# Autodesk Inventor assembly: 射出_骨組み
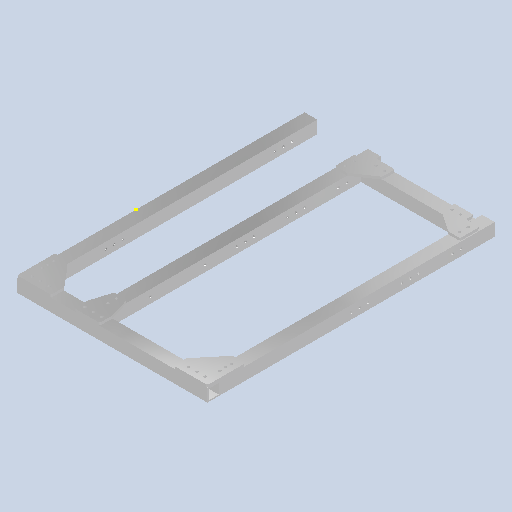
[picture p0: Inventor's stored thumbnail of the model, 512x512]
Saved by Autodesk Inventor 2023 (Build 270158000, 158)
## iProperties
Created: 2022-04-24
Part Number: 射出_骨組み
Document SubType Name: Assembly
Designer: yuta
Author: yuta
## Documents named in this file (9)
- C:\Users\yuta\Documents\NHK\射出_骨組み.iam
- C:\Users\yuta\Documents\NHK\射出_角柱2.ipt
- C:\Users\yuta\Documents\NHK\射出_角柱5.ipt
- C:\Users\yuta\Documents\NHK\射出_角柱4.ipt
- C:\Users\yuta\Documents\NHK\射出_角柱3.ipt
- C:\Users\yuta\Documents\NHK\射出_固定3.ipt
- C:\Users\yuta\Documents\NHK\射出_固定5.ipt
- C:\Users\yuta\Documents\NHK\射出_固定4.ipt
- C:\Users\yuta\Documents\NHK\射出_角柱9.ipt
## Components (10 placed, 8 different names)
1. 射出_角柱2:1 — メイト:18, メイト:19, メイト:20, メイト:21, メイト:25, メイト:26, メイト:27
2. 射出_角柱5:1 — メイト:14, メイト:15, フラッシュ:3, メイト:16, メイト:17, フラッシュ:4
3. 射出_角柱4:1 — メイト:1, フラッシュ:1, フラッシュ:2, メイト:5, メイト:6, メイト:22, メイト:23, メイト:24, メイト:29
4. 射出_角柱3:1 — メイト:1, フラッシュ:1, フラッシュ:2, メイト:2, メイト:3, メイト:4, メイト:7, メイト:8, メイト:9, メイト:10, メイト:11, メイト:12, メイト:13, メイト:15, フラッシュ:4, メイト:19
5. 射出_固定3:1 — メイト:11, メイト:12, メイト:13, メイト:14, フラッシュ:3, メイト:16, メイト:17
6. 射出_固定3:2 — メイト:2, メイト:3, メイト:4, メイト:5, メイト:6
7. 射出_固定5:1 — メイト:7, メイト:8, メイト:9, メイト:10, メイト:18, メイト:20, メイト:21
8. 射出_固定4:1 — メイト:22, メイト:23, メイト:24, メイト:28, メイト:30, メイト:31
9. 射出_固定4:2 — メイト:25, メイト:26, メイト:27, メイト:32, メイト:33
10. 射出_角柱9:1 — メイト:28, メイト:29, メイト:30, メイト:31, メイト:32, メイト:33
## Relationships (37: Mate 33, Flush 4)
- メイト:1 [Mate]: 射出_角柱4:1 ↔ 射出_角柱3:1
- フラッシュ:1 [Flush]: 射出_角柱4:1 ↔ 射出_角柱3:1
- フラッシュ:2 [Flush]: 射出_角柱4:1 ↔ 射出_角柱3:1
- メイト:2 [Mate]: 射出_角柱3:1 ↔ 射出_固定3:2
- メイト:3 [Mate]: 射出_角柱3:1 ↔ 射出_固定3:2
- メイト:4 [Mate]: 射出_角柱3:1 ↔ 射出_固定3:2
- メイト:5 [Mate]: 射出_角柱4:1 ↔ 射出_固定3:2
- メイト:6 [Mate]: 射出_角柱4:1 ↔ 射出_固定3:2
- メイト:7 [Mate]: 射出_角柱3:1 ↔ 射出_固定5:1
- メイト:8 [Mate]: 射出_角柱3:1 ↔ 射出_固定5:1
- メイト:9 [Mate]: 射出_角柱3:1 ↔ 射出_固定5:1
- メイト:10 [Mate]: 射出_角柱3:1 ↔ 射出_固定5:1
- メイト:11 [Mate]: 射出_角柱3:1 ↔ 射出_固定3:1
- メイト:12 [Mate]: 射出_角柱3:1 ↔ 射出_固定3:1
- メイト:13 [Mate]: 射出_角柱3:1 ↔ 射出_固定3:1
- メイト:14 [Mate]: 射出_角柱5:1 ↔ 射出_固定3:1
- メイト:15 [Mate]: 射出_角柱5:1 ↔ 射出_角柱3:1
- フラッシュ:3 [Flush]: 射出_角柱5:1 ↔ 射出_固定3:1
- メイト:16 [Mate]: 射出_角柱5:1 ↔ 射出_固定3:1
- メイト:17 [Mate]: 射出_角柱5:1 ↔ 射出_固定3:1
- フラッシュ:4 [Flush]: 射出_角柱5:1 ↔ 射出_角柱3:1
- メイト:18 [Mate]: 射出_角柱2:1 ↔ 射出_固定5:1
- メイト:19 [Mate]: 射出_角柱2:1 ↔ 射出_角柱3:1
- メイト:20 [Mate]: 射出_角柱2:1 ↔ 射出_固定5:1
- メイト:21 [Mate]: 射出_角柱2:1 ↔ 射出_固定5:1
- メイト:22 [Mate]: 射出_角柱4:1 ↔ 射出_固定4:1
- メイト:23 [Mate]: 射出_角柱4:1 ↔ 射出_固定4:1
- メイト:24 [Mate]: 射出_角柱4:1 ↔ 射出_固定4:1
- メイト:25 [Mate]: 射出_角柱2:1 ↔ 射出_固定4:2
- メイト:26 [Mate]: 射出_角柱2:1 ↔ 射出_固定4:2
- メイト:27 [Mate]: 射出_角柱2:1 ↔ 射出_固定4:2
- メイト:28 [Mate]: 射出_固定4:1 ↔ 射出_角柱9:1
- メイト:29 [Mate]: 射出_角柱4:1 ↔ 射出_角柱9:1
- メイト:30 [Mate]: 射出_固定4:1 ↔ 射出_角柱9:1
- メイト:31 [Mate]: 射出_固定4:1 ↔ 射出_角柱9:1
- メイト:32 [Mate]: 射出_固定4:2 ↔ 射出_角柱9:1
- メイト:33 [Mate]: 射出_固定4:2 ↔ 射出_角柱9:1
